# Autodesk Inventor assembly: headstage+flex connector
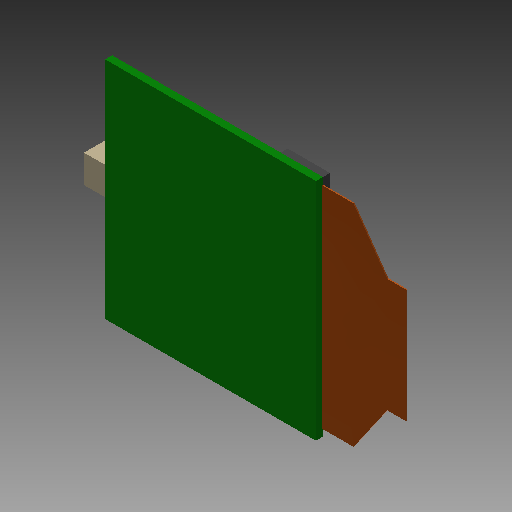
[picture p0: Inventor's stored thumbnail of the model, 512x512]
Saved by Autodesk Inventor 2019 (Build 230136000, 136)
## iProperties
Created: 2020-03-27
Part Number: headstage+flex connector
Document SubType Name: Assembly
Designer: Thomas Zhihao Luo
Author: Thomas Zhihao Luo
## Documents named in this file (3)
- C:\Users\Thomas Zhihao Luo\Documents\chronic_neuropixels\2.611\headstage+flex connector.iam
- C:\Users\Thomas Zhihao Luo\Documents\chronic_neuropixels\2.611\headstage.ipt
- C:\Users\Thomas Zhihao Luo\Documents\chronic_neuropixels\2.611\flexcable3.ipt
## Components (2 placed, 2 different names)
1. headstage:1
2. flexcable3:1
## Relationships (1: WeldJoint 1)
- [WeldJoint]: headstage:1 ↔ flexcable3:1
